# Autodesk Inventor assembly: Horizontal Leg Test v3.1
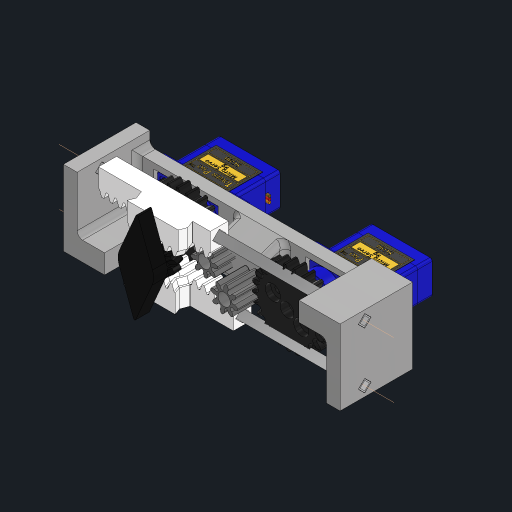
[picture p0: Inventor's stored thumbnail of the model, 512x512]
Saved by Autodesk Inventor 2023.2 (Build 272271030, 271C)
## iProperties
Created: 2023-11-19
Part Number: Horizontal Leg Test v3.1
Document SubType Name: Assembly
Designer: robpl
Author: robpl
## Documents named in this file (10)
- C:\Users\robpl\OneDrive\Documents\Arduino\Onslaught\CAD\Horizontal Leg Test\Horizontal Leg Test v3.1.iam
- C:\Users\robpl\OneDrive\Documents\Arduino\Onslaught\CAD\Horizontal Leg Test\Horizontal Leg Test v3\Frame V3.1.ipt
- C:\Users\robpl\OneDrive\Documents\Arduino\Onslaught\CAD\Horizontal Leg Test\SG90 - Micro Servo 9g - Tower Pro.ipt
- C:\Users\robpl\OneDrive\Documents\Arduino\Onslaught\CAD\Horizontal Leg Test\Horizontal Leg Test v3\Design Accelerator\Spur Gears3.iam
- C:\Users\robpl\OneDrive\Documents\Arduino\Onslaught\CAD\Horizontal Leg Test\Horizontal Leg Test v3\Intermediate Gear.ipt
- C:\Users\robpl\OneDrive\Documents\Arduino\Onslaught\CAD\Horizontal Leg Test\Horizontal Leg Test v3\Servo Gear V3.1.ipt
- C:\Users\robpl\OneDrive\Documents\Arduino\Onslaught\CAD\Horizontal Leg Test\Horizontal Leg Test v3\Rack Rail v3.ipt
- C:\Users\robpl\OneDrive\Documents\Arduino\Onslaught\CAD\Horizontal Leg Test\Horizontal Leg Test v3\Rack.ipt
- C:\Users\robpl\OneDrive\Documents\Arduino\Onslaught\CAD\Horizontal Leg Test\Horizontal Leg Test v3\Leg.ipt
- C:\Users\robpl\OneDrive\Documents\Arduino\Onslaught\CAD\Horizontal Leg Test\Horizontal Leg Test v3\M2 Knurled Nut.ipt
## Components (15 placed, 9 different names)
1. Frame V3.1:1 — Mate:1, Mate:2, Mate:5, Mate:6, Mate:7, Mate:8, Mate:9, Mate:11, Mate:12, Angle:2, Mate:21, Mate:22, Mate:25, Mate:26, Mate:27, Mate:28, Mate:29, Flush:1, Angle:3, Mate:30, Mate:31, Flush:2, Mate:32
2. SG90 - Micro Servo 9g - Tower Pro:1 — Mate:1, Mate:5, Mate:6, Mate:15, Mate:16
3. SG90 - Micro Servo 9g - Tower Pro:2 — Mate:2, Mate:7, Mate:8, Mate:13, Flush:3
4. Spur Gears:1 [sub-assembly]
5. Intermediate Gear:1 — Mate:9, Rotation:1, Rotation/Translation:2, Flush:4
6. Intermediate Gear:2 — Mate:11, Mate:12, Rotation:2, Rotation/Translation:1
7. Servo Gear V3.1:1 — Mate:13, Rotation:1, Flush:3, Flush:4
8. Servo Gear V3.1:2 — Mate:15, Mate:16, Rotation:2
9. Rack Rail v3:1 — Mate:31, Flush:2
10. Rack Rail v3:2 — Mate:29, Flush:1, Angle:3
11. Rack:1 — Angle:1, Angle:2, Mate:22, Mate:23, Rotation/Translation:2, Mate:30
12. Rack:2 — Angle:1, Mate:21, Rotation/Translation:1, Mate:32
13. Leg:1 — Mate:23, Mate:24
14. M2 Knurled Nut:1 — Mate:25, Mate:27
15. M2 Knurled Nut:2 — Mate:26, Mate:28
## Relationships (35: Mate 24, Flush 4, Angle 3, RelateRotation 2, RelateRotateTranslate 2)
- Mate:1: Frame V3.1:1 ↔ SG90 - Micro Servo 9g - Tower Pro:1
- Mate:2: Frame V3.1:1 ↔ SG90 - Micro Servo 9g - Tower Pro:2
- Mate:5: Frame V3.1:1 ↔ SG90 - Micro Servo 9g - Tower Pro:1
- Mate:6: Frame V3.1:1 ↔ SG90 - Micro Servo 9g - Tower Pro:1
- Mate:7: Frame V3.1:1 ↔ SG90 - Micro Servo 9g - Tower Pro:2
- Mate:8: Frame V3.1:1 ↔ SG90 - Micro Servo 9g - Tower Pro:2
- Mate:9: Frame V3.1:1 ↔ Intermediate Gear:1
- Mate:11: Frame V3.1:1 ↔ Intermediate Gear:2
- Mate:12 (0.5 mm): Frame V3.1:1 ↔ Intermediate Gear:2
- Mate:13: SG90 - Micro Servo 9g - Tower Pro:2 ↔ Servo Gear V3.1:1
- Mate:15: SG90 - Micro Servo 9g - Tower Pro:1 ↔ Servo Gear V3.1:2
- Mate:16: SG90 - Micro Servo 9g - Tower Pro:1 ↔ Servo Gear V3.1:2
- Angle:1 (180 deg): Rack:1 ↔ Rack:2
- Angle:2 (0 deg): Frame V3.1:1 ↔ Rack:1
- Mate:21: Frame V3.1:1 ↔ Rack:2
- Mate:22: Frame V3.1:1 ↔ Rack:1
- Mate:23 (-4.75 mm): Rack:1 ↔ Leg:1
- Mate:24: Leg:1
- Rotation:1 [RelateRotation] (0.32 ul): Intermediate Gear:1 ↔ Servo Gear V3.1:1
- Rotation:2 [RelateRotation] (3.125 ul): Intermediate Gear:2 ↔ Servo Gear V3.1:2
- Rotation/Translation:1 [RelateRotateTranslate] (25.1327 mm): Intermediate Gear:2 ↔ Rack:2
- Rotation/Translation:2 [RelateRotateTranslate] (25.1327 mm): Intermediate Gear:1 ↔ Rack:1
- Mate:25: Frame V3.1:1 ↔ M2 Knurled Nut:1
- Mate:26: Frame V3.1:1 ↔ M2 Knurled Nut:2
- Mate:27: Frame V3.1:1 ↔ M2 Knurled Nut:1
- Mate:28: Frame V3.1:1 ↔ M2 Knurled Nut:2
- Mate:29: Frame V3.1:1 ↔ Rack Rail v3:2
- Flush:1: Frame V3.1:1 ↔ Rack Rail v3:2
- Angle:3 (0 deg): Frame V3.1:1 ↔ Rack Rail v3:2
- Mate:30: Frame V3.1:1 ↔ Rack:1
- Mate:31: Frame V3.1:1 ↔ Rack Rail v3:1
- Flush:2: Frame V3.1:1 ↔ Rack Rail v3:1
- Mate:32: Frame V3.1:1 ↔ Rack:2
- Flush:3 (-0.5 mm): SG90 - Micro Servo 9g - Tower Pro:2 ↔ Servo Gear V3.1:1
- Flush:4: Intermediate Gear:1 ↔ Servo Gear V3.1:1
